# Autodesk Inventor assembly: C
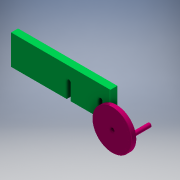
[picture p0: Inventor's stored thumbnail of the model, 180x180]
Saved by Autodesk Inventor 2019 (Build 230136000, 136)
## iProperties
Created: 2020-03-27
Part Number: C
Document SubType Name: Assembly
Designer: Pulag
Author: Pulag
## Documents named in this file (3)
- C:\Users\Pulag\Documents\GitHub\24th_TDK_Project_D5\CAD\frame\日內瓦機構\C.iam
- C:\Users\Pulag\Documents\GitHub\24th_TDK_Project_D5\CAD\frame\C1.ipt
- C:\Users\Pulag\Documents\GitHub\24th_TDK_Project_D5\CAD\frame\日內瓦機構\C2.ipt
## Components (2 placed, 2 different names)
1. C1:1 — Flush:1, Mate:1, Mate:3
2. C2:1 — Flush:1, Mate:4
## Relationships (4: Mate 3, Flush 1)
- Flush:1: C1:1 ↔ C2:1
- Mate:1: C1:1
- Mate:3: C1:1
- Mate:4: C2:1
